# Autodesk Inventor assembly: Tipo BLE Assembly
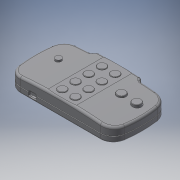
[picture p0: Inventor's stored thumbnail of the model, 180x180]
Saved by Autodesk Inventor 2019 (Build 230136000, 136)
## iProperties
Created: 2020-02-19
Part Number: Tipo BLE Assembly
Document SubType Name: Assembly
Designer: Vijay
Author: Vijay
## Documents named in this file (8)
- C:\Users\Vijay\Documents\CAD Files\Tipo\Tipo BLE Assembly.iam
- C:\Users\Vijay\Documents\CAD Files\Tipo\Clampshell Body Top.ipt
- C:\Users\Vijay\Documents\CAD Files\Tipo\Omron 12x12 button (1).ipt
- C:\Users\Vijay\Documents\CAD Files\Tipo\Button Head.ipt
- C:\Users\Vijay\Documents\CAD Files\Tipo\joystick.ipt
- C:\Users\Vijay\Documents\CAD Files\Tipo\ESP.ipt
- C:\Users\Vijay\Documents\CAD Files\Tipo\perfboard.ipt
- C:\Users\Vijay\Documents\CAD Files\Tipo\back cover.ipt
## Components (25 placed, 7 different names)
1. Clampshell Body Top:1 — Mate:15, Mate:16, Mate:17, Mate:18, Mate:19, Mate:20, Mate:21, Mate:24, Angle:2, Flush:8, Flush:14
2. Omron 12x12 button (1):1 — Mate:1, Mate:2, Angle:8
3. Button Head:1 — Mate:1, Mate:2, Mate:15, Flush:1, Flush:2
4. Omron 12x12 button (1):2 — Angle:4, Angle:8
5. Button Head:2 — Mate:17, Flush:2, Flush:3
6. Omron 12x12 button (1):3 — Angle:7
7. Button Head:3 — Mate:18, Flush:5
8. Omron 12x12 button (1):4 — Angle:3, Angle:4
9. Button Head:4 — Mate:19, Flush:3, Flush:4, Flush:7
10. Omron 12x12 button (1):5 — Angle:5
11. Button Head:5 — Mate:20, Flush:4, Flush:5, Flush:6
12. Omron 12x12 button (1):6 — Angle:2, Angle:3, Angle:5, Angle:6
13. Button Head:6 — Mate:21, Flush:7, Flush:8
14. Omron 12x12 button (1):7 — Angle:7
15. Button Head:7 — Mate:16, Flush:1, Flush:12
16. Omron 12x12 button (1):8 — Angle:6, Flush:9
17. Button Head:8 — Mate:24, Flush:6
18. joystick:1 — Flush:9
19. Omron 12x12 button (1):9 — Flush:11
20. Button Head:9 — Flush:10
21. Omron 12x12 button (1):10 — Flush:11, Flush:13
22. Button Head:10 — Flush:10, Flush:12
23. ESP:1 — Mate:29
24. perfboard:1 — Flush:13, Mate:29
25. back cover:1 — Flush:14
## Relationships (50: Mate 29, Flush 14, Angle 7)
- Mate:1: Omron 12x12 button (1):1 ↔ Button Head:1
- Mate:2 (3 mm): Omron 12x12 button (1):1 ↔ Button Head:1
- [Mate]: Omron 12x12 button (1):2 ↔ Button Head:2
- [Mate] (3 mm): Omron 12x12 button (1):2 ↔ Button Head:2
- [Mate]: Omron 12x12 button (1):3 ↔ Button Head:3
- [Mate] (3 mm): Omron 12x12 button (1):3 ↔ Button Head:3
- [Mate]: Omron 12x12 button (1):4 ↔ Button Head:4
- [Mate] (3 mm): Omron 12x12 button (1):4 ↔ Button Head:4
- [Mate]: Omron 12x12 button (1):5 ↔ Button Head:5
- [Mate] (3 mm): Omron 12x12 button (1):5 ↔ Button Head:5
- [Mate]: Omron 12x12 button (1):6 ↔ Button Head:6
- [Mate] (3 mm): Omron 12x12 button (1):6 ↔ Button Head:6
- [Mate]: Omron 12x12 button (1):7 ↔ Button Head:7
- [Mate] (3 mm): Omron 12x12 button (1):7 ↔ Button Head:7
- Mate:15: Clampshell Body Top:1 ↔ Button Head:1
- Mate:16: Clampshell Body Top:1 ↔ Button Head:7
- Mate:17: Clampshell Body Top:1 ↔ Button Head:2
- Mate:18: Clampshell Body Top:1 ↔ Button Head:3
- Mate:19: Clampshell Body Top:1 ↔ Button Head:4
- Mate:20: Clampshell Body Top:1 ↔ Button Head:5
- Mate:21: Clampshell Body Top:1 ↔ Button Head:6
- [Mate]: Omron 12x12 button (1):8 ↔ Button Head:8
- [Mate] (3 mm): Omron 12x12 button (1):8 ↔ Button Head:8
- Mate:24: Clampshell Body Top:1 ↔ Button Head:8
- Flush:1: Button Head:1 ↔ Button Head:7
- Flush:2: Button Head:1 ↔ Button Head:2
- Flush:3: Button Head:2 ↔ Button Head:4
- Flush:4: Button Head:4 ↔ Button Head:5
- Flush:5: Button Head:3 ↔ Button Head:5
- Flush:6: Button Head:5 ↔ Button Head:8
- Flush:7: Button Head:4 ↔ Button Head:6
- Angle:2 (0 deg): Clampshell Body Top:1 ↔ Omron 12x12 button (1):6
- Angle:3 (0 deg): Omron 12x12 button (1):4 ↔ Omron 12x12 button (1):6
- Angle:4 (0 deg): Omron 12x12 button (1):2 ↔ Omron 12x12 button (1):4
- Angle:5 (0 deg): Omron 12x12 button (1):5 ↔ Omron 12x12 button (1):6
- Angle:6 (0 deg): Omron 12x12 button (1):6 ↔ Omron 12x12 button (1):8
- Angle:7 (0 deg): Omron 12x12 button (1):3 ↔ Omron 12x12 button (1):7
- Angle:8 (0 deg): Omron 12x12 button (1):1 ↔ Omron 12x12 button (1):2
- Flush:8 (-1 mm): Clampshell Body Top:1 ↔ Button Head:6
- Flush:9: Omron 12x12 button (1):8 ↔ joystick:1
- [Mate]: Omron 12x12 button (1):9 ↔ Button Head:9
- [Mate] (3 mm): Omron 12x12 button (1):9 ↔ Button Head:9
- [Mate]: Omron 12x12 button (1):10 ↔ Button Head:10
- [Mate] (3 mm): Omron 12x12 button (1):10 ↔ Button Head:10
- Flush:10: Button Head:9 ↔ Button Head:10
- Flush:11: Omron 12x12 button (1):9 ↔ Omron 12x12 button (1):10
- Flush:12: Button Head:7 ↔ Button Head:10
- Flush:13: Omron 12x12 button (1):10 ↔ perfboard:1
- Mate:29: ESP:1 ↔ perfboard:1
- Flush:14: Clampshell Body Top:1 ↔ back cover:1
## Named parameters: d3_d1 = 0 mm, d4_d2 = 3 mm, d5_d1 = 0 mm, d6_d2 = 3 mm, d7_d1 = 0 mm, d8_d2 = 3 mm, d9_d1 = 0 mm, d10_d2 = 3 mm, d11_d1 = 0 mm, d12_d2 = 3 mm, d13_d1 = 0 mm, d14_d2 = 3 mm, d22_d1 = 0 mm, d23_d2 = 3 mm, d44_d13_d1 = 0 mm, d45_d14_d2 = 3 mm, d46_d44_d13_d1 = 0 mm, d47_d45_d14_d2 = 3 mm
